# Autodesk Inventor assembly: WheelWithPulley
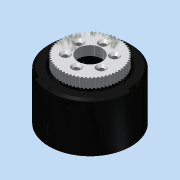
[picture p0: Inventor's stored thumbnail of the model, 180x180]
Saved by Autodesk Inventor 2015 (Build 190159000, 159)
## iProperties
Created: 2015-11-06
Part Number: WheelWithPulley
Document SubType Name: Assembly
Designer: Raphael
Author: Raphael
## Documents named in this file (4)
- \\psf\Home\Documents\electric-skateboard\CAD\WheelWithPulley.iam
- \\psf\Home\Documents\electric-skateboard\CAD\WheelWithBearing.iam
- \\psf\Home\Documents\electric-skateboard\CAD\WheelPulleyAssembly.iam
- \\psf\Home\Documents\electric-skateboard\CAD\WheelInsertOuter.ipt
## Components (3 placed, 3 different names)
1. WheelWithBearing:1 [sub-assembly] — Mate:1, Mate:3, Mate:5
2. WheelPulleyAssembly:1 [sub-assembly] — Mate:1, Mate:4
3. WheelInsertOuter:1 — Mate:3, Mate:4, Mate:5
## Relationships (4: Mate 4)
- Mate:1: WheelWithBearing:1 ↔ WheelPulleyAssembly:1
- Mate:3: WheelWithBearing:1 ↔ WheelInsertOuter:1
- Mate:4: WheelPulleyAssembly:1 ↔ WheelInsertOuter:1
- Mate:5: WheelWithBearing:1 ↔ WheelInsertOuter:1
